# Autodesk Inventor assembly: 揺動節+ヘッケン
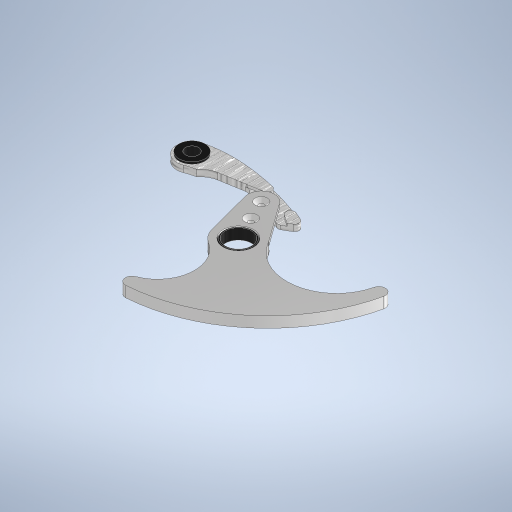
[picture p0: Inventor's stored thumbnail of the model, 512x512]
Saved by Autodesk Inventor 2023 (Build 270158000, 158)
## iProperties
Created: 2022-01-08
Part Number: 揺動節+ヘッケン
Document SubType Name: Assembly
Designer: acps
Author: acps
## Documents named in this file (7)
- C:\Users\muzho\Documents\srdc\srdc_2\脚\揺動節+ヘッケン.iam
- C:\Users\muzho\Documents\srdc\srdc_2\脚\揺動節.ipt
- C:\Users\muzho\Documents\srdc\srdc_2\脚\ヘッケン.ipt
- C:\Users\muzho\Documents\srdc\srdc_2\脚\ヘッケン抑え.ipt
- C:\Users\muzho\Documents\srdc\srdc_2\オイレス\w5f12-14n.ipt
- C:\Users\muzho\Documents\srdc\srdc_2\オイレス\w1.5f5-7n.ipt
- C:\Users\muzho\Documents\srdc\srdc_2\オイレス\w5f6-12a.ipt
## Components (6 placed, 6 different names)
1. 揺動節:1 — Insert:5, Insert:6
2. ヘッケン:1 — Mate:1, Mate:2, Insert:6, Insert:7, Insert:8, Insert:9
3. ヘッケン抑え:1 — Mate:1, Mate:2, Insert:8
4. w5f12-14n:1 — Insert:9
5. w1.5f5-7n:1 — Insert:7
6. w5f6-12a:1 — Insert:5
## Relationships (7: Insert 5, Mate 2)
- Insert:5: 揺動節:1 ↔ w5f6-12a:1
- Mate:1: ヘッケン:1 ↔ ヘッケン抑え:1
- Mate:2: ヘッケン:1 ↔ ヘッケン抑え:1
- Insert:6: 揺動節:1 ↔ ヘッケン:1
- Insert:7: ヘッケン:1 ↔ w1.5f5-7n:1
- Insert:8: ヘッケン:1 ↔ ヘッケン抑え:1
- Insert:9: ヘッケン:1 ↔ w5f12-14n:1
